# Autodesk Inventor assembly: Base link
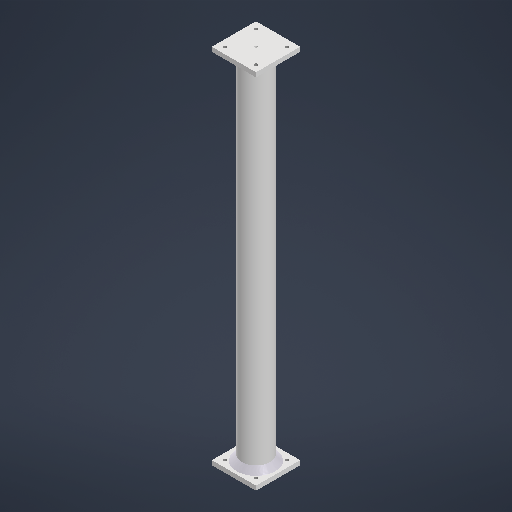
[picture p0: Inventor's stored thumbnail of the model, 512x512]
Saved by Autodesk Inventor 2026.3 (Build 303398000, 398)
## iProperties
Created: 2026-07-28
Part Number: Base link
Document SubType Name: Weldment
Designer: matot
Weld Material: Aluminum 6061, Welded
Author: matot
## Documents named in this file (3)
- C:\Users\matot\OneDrive - Stellenbosch University\2026\MechatronicsProject478\Building the joint\Joint Assembly\Base link.iam
- C:\Users\matot\OneDrive - Stellenbosch University\2026\MechatronicsProject478\Building the joint\Joint Assembly\Bottom link plate.ipt
- C:\Users\matot\OneDrive - Stellenbosch University\2026\MechatronicsProject478\Building the joint\Joint Assembly\Bottom link body.ipt
## Components (3 placed, 2 different names)
1. Bottom link plate:2 — Insert:1
2. Bottom link plate:3 — Insert:2
3. Bottom link body:1 — Insert:1, Insert:2
## Relationships (2: Insert 2)
- Insert:1: Bottom link plate:2 ↔ Bottom link body:1
- Insert:2: Bottom link plate:3 ↔ Bottom link body:1
